# Autodesk Inventor assembly: M178-PHTM-4000
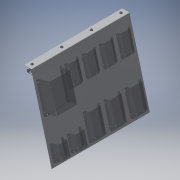
[picture p0: Inventor's stored thumbnail of the model, 180x180]
Saved by Autodesk Inventor 2018 (Build 220105000, 105)
## iProperties
Created: 2004-11-29
Part Number: M178-PHTM-4000
Document SubType Name: Assembly
Designer: Autodesk, Inc.
Manufacturer: Standard
Standards Organization: Custom
Mass: 1631.03 g
Surface Area: 9213.9 cm^2
Volume: 761.257 cm^3
Density: 2.14255 g/cm^3
CAGE: 1LJX3
Dept. ID: Product Design
Description #2: ---
Finish #1: ---
Finish #2: ---
Material ID: ---
Project Number: ---
Author: Autodesk, Inc.
## Documents named in this file (7)
- C:\Autodesk\autodesk_inventor_2017_samples\Models\Assemblies\Test Station\Components\M178-4000 Phantom.iam
- C:\Autodesk\autodesk_inventor_2017_samples\Models\Assemblies\Test Station\Components\M178-4000.iam
- C:\Autodesk\autodesk_inventor_2017_samples\Models\Assemblies\Test Station\Components\24-112-8.ipt
- C:\Autodesk\autodesk_inventor_2017_samples\Models\Assemblies\Test Station\Components\24-116-8.ipt
- C:\Autodesk\autodesk_inventor_2017_samples\Models\Assemblies\Test Station\Components\20-058.ipt
- C:\Users\kelleyb.ADS\Desktop\Samples MIGRATED 2009 224 RTM_1\Standard Parts\Test Station Content\Fastners\2X-YYY-ZZ IPS Screws.ipt
- C:\Users\kelleyb.ADS\Desktop\Samples MIGRATED 2009 224 RTM_1\Standard Parts\Test Station Content\Fastners\20-XXX TSlot Nuts.ipt
## Components (13 placed, 4 different names)
1. M178-4000:1 [sub-assembly] — Insert:1, Mate:3, Angle:1
2. 24-112-8:1 — Insert:1, Mate:1
3. 20-058:1 — Mate:1, Mate:3, Angle:1
4. 24-112-8:2
5. 20-058:3
6. 24-112-8:3
7. 20-058:4
8. 24-112-8:4
9. 20-058:5
10. 20-058:2 — Mate:2
11. 24-116-8:5 — Mate:2
12. 20-058:6
13. 24-116-8:6
## Component patterns: (4 elements, first: 24-112-8:1 + 20-058:1), (2 elements, first: 20-058:2 + 24-116-8:5)
## Relationships (5: Mate 3, Insert 1, Angle 1)
- Insert:1: M178-4000:1 ↔ 24-112-8:1
- Mate:1: 24-112-8:1 ↔ 20-058:1
- Mate:2: 20-058:2 ↔ 24-116-8:5
- Mate:3 (4.5 mm): M178-4000:1 ↔ 20-058:1
- Angle:1 (0 deg): M178-4000:1 ↔ 20-058:1
